# Autodesk Inventor assembly: fan_holder_0130
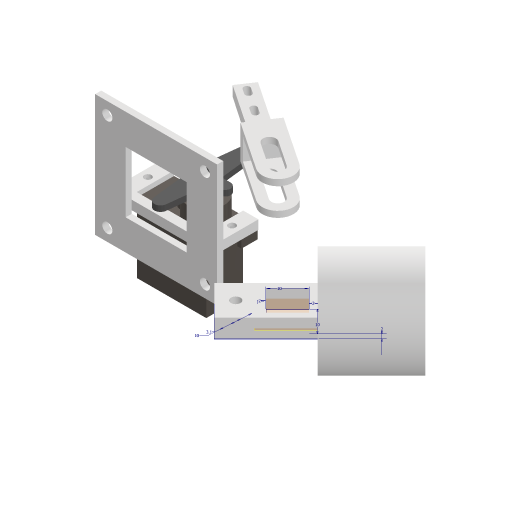
[picture p0: Inventor's stored thumbnail of the model, 512x512]
Saved by Autodesk Inventor 2024 (Build 280153000, 153)
## iProperties
Created: 2024-01-30
Part Number: fan_holder_0130
Document SubType Name: Assembly
Designer: admin
Author: admin
## Documents named in this file (6)
- C:\Users\admin\OneDrive\文件\碩士研究\prototype\fan_holder_0227\fan_holder_0227.iam
- C:\Users\admin\OneDrive\文件\碩士研究\prototype\fan_holder_0227\elemagnetic.ipt
- C:\Users\admin\OneDrive\文件\碩士研究\prototype\fan_holder_0227\elemagnetic_holder_0306.ipt
- C:\Users\admin\OneDrive\文件\碩士研究\prototype\fan_holder_0227\fan_holder_0301.ipt
- C:\Users\admin\OneDrive\文件\碩士研究\prototype\fan_holder_0227\SG90_holder_0213.ipt
- C:\Users\admin\Downloads\mg90s-servo-2.snapshot.1\MG90S Servo-All\MG90S Servo-All.iam
## Components (5 placed, 5 different names)
1. elemagnetic:1 — 貼合:9, 貼合:10
2. elemagnetic_holder_0306:1 — 貼合:9, 貼合:10, 貼合:11, 貼合:12, 角度:1
3. fan_holder_0301:1 — 貼合:11, 貼合:12
4. SG90_holder_0213:1 — 角度:1, 貼合:13, 貼合:14, 貼合:15
5. MG90S Servo-All:1 [sub-assembly] — 貼合:13, 貼合:14, 貼合:15
## Relationships (8: Mate 7, Angle 1)
- 貼合:9 [Mate]: elemagnetic:1 ↔ elemagnetic_holder_0306:1
- 貼合:10 [Mate]: elemagnetic:1 ↔ elemagnetic_holder_0306:1
- 貼合:11 [Mate]: elemagnetic_holder_0306:1 ↔ fan_holder_0301:1
- 貼合:12 [Mate]: elemagnetic_holder_0306:1 ↔ fan_holder_0301:1
- 角度:1 [Angle] (135 deg): elemagnetic_holder_0306:1 ↔ SG90_holder_0213:1
- 貼合:13 [Mate]: SG90_holder_0213:1 ↔ MG90S Servo-All:1
- 貼合:14 [Mate]: SG90_holder_0213:1 ↔ MG90S Servo-All:1
- 貼合:15 [Mate]: SG90_holder_0213:1 ↔ MG90S Servo-All:1
